# Autodesk Inventor assembly: Foot
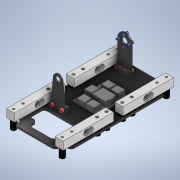
[picture p0: Inventor's stored thumbnail of the model, 180x180]
Saved by Autodesk Inventor 2022.3 (Build 263350000, 350)
## iProperties
Created: 2022-06-04
Part Number: Foot
Document SubType Name: Assembly
Designer: Masato Kubotera
Author: Masato Kubotera
## Documents named in this file (10)
- C:\Users\Masato\Documents\Inventor\CIT Brains\SUSTAINA-OP - mod\LowerBody\Foot\Foot.iam
- C:\Users\Masato\Documents\Inventor\CIT Brains\SUSTAINA-OP - mod\LowerBody\Foot\Foot_back_frame.ipt
- C:\Users\Masato\Documents\Inventor\CIT Brains\SUSTAINA-OP - mod\LowerBody\Foot\Foot_front_frame.ipt
- C:\Users\Masato\Documents\Inventor\CIT Brains\SUSTAINA-OP - mod\LowerBody\Foot\Foot_root_block.ipt
- C:\Users\Masato\Documents\Inventor\CIT Brains\SUSTAINA-OP - mod\LowerBody\Foot\Sole_frame.ipt
- C:\Users\Masato\Documents\Inventor\CIT Brains\SUSTAINA-OP - mod\ReadyMade\Screw\UC-0308.ipt
- C:\Users\Masato\Documents\Inventor\CIT Brains\SUSTAINA-OP - mod\ReadyMade\Screw\UC-2606.ipt
- C:\Users\Masato\Documents\Inventor\CIT Brains\SUSTAINA-OP - mod\LowerBody\Foot\LoadCell_unit.iam
- C:\Users\Masato\Documents\Inventor\CIT Brains\SUSTAINA-OP - mod\ReadyMade\Screw\FC-0515EB.ipt
- C:\Users\Masato\Documents\Inventor\CIT Brains\SUSTAINA-OP - mod\ReadyMade\ElectronicComponents\Quad-Load-Cell-Amplifier-to-RS-485-Conv-Module.ipt
## Components (30 placed, 9 different names)
1. Sole_frame:1 — 挿入:1, 挿入:2, 挿入:3, 挿入:4, 挿入:13, 挿入:14, 挿入:15, 挿入:16, 挿入:33, 挿入:34, 挿入:35, 挿入:36, 挿入:37, 挿入:38, 挿入:39, 挿入:40, 挿入:41, 挿入:42, 挿入:43, 挿入:44, 挿入:45, 挿入:46, 挿入:47, 挿入:48, 挿入:49, 挿入:50
2. Foot_front_frame:1 — 挿入:5, 挿入:6, メイト:1, メイト:2, 挿入:31, 挿入:32
3. Foot_back_frame:1 — 挿入:7, 挿入:8, 挿入:17, 挿入:18, 挿入:19, 挿入:20, 挿入:29, 挿入:30
4. Foot_root_block:1 — 挿入:1, 挿入:2, 挿入:5, 挿入:6
5. Foot_root_block:2 — 挿入:3, 挿入:4, 挿入:7, 挿入:8
6. UC-0308:5 — 挿入:32
7. UC-0308:6 — 挿入:31
8. UC-0308:7 — 挿入:29
9. UC-0308:8 — 挿入:30
10. UC-0308:1 — 挿入:13
11. UC-0308:2 — 挿入:14
12. UC-0308:3 — 挿入:15
13. UC-0308:4 — 挿入:16
14. UC-2606:1 — 挿入:17
15. UC-2606:2 — 挿入:18
16. UC-2606:3 — 挿入:19
17. UC-2606:4 — 挿入:20
18. LoadCell_unit:1 [sub-assembly] — 挿入:33, 挿入:34
19. LoadCell_unit:2 [sub-assembly] — 挿入:35, 挿入:36
20. LoadCell_unit:3 [sub-assembly] — 挿入:37, 挿入:38
21. LoadCell_unit:4 [sub-assembly] — 挿入:39, 挿入:40
22. FC-0515EB:1 — 挿入:41
23. FC-0515EB:2 — 挿入:42
24. FC-0515EB:3 — 挿入:43
25. FC-0515EB:4 — 挿入:44
26. FC-0515EB:5 — 挿入:45
27. FC-0515EB:6 — 挿入:46
28. FC-0515EB:7 — 挿入:47
29. FC-0515EB:8 — 挿入:48
30. Quad-Load-Cell-Amplifier-to-RS-485-Conv-Module:1 — 挿入:49, 挿入:50
## Relationships (40: Insert 38, Mate 2)
- メイト:1 [Mate]: Foot_front_frame:1
- メイト:2 [Mate]: Foot_front_frame:1
- 挿入:1 [Insert]: Sole_frame:1 ↔ Foot_root_block:1
- 挿入:2 [Insert]: Sole_frame:1 ↔ Foot_root_block:1
- 挿入:3 [Insert]: Sole_frame:1 ↔ Foot_root_block:2
- 挿入:4 [Insert]: Sole_frame:1 ↔ Foot_root_block:2
- 挿入:5 [Insert]: Foot_front_frame:1 ↔ Foot_root_block:1
- 挿入:6 [Insert]: Foot_front_frame:1 ↔ Foot_root_block:1
- 挿入:7 [Insert]: Foot_back_frame:1 ↔ Foot_root_block:2
- 挿入:8 [Insert]: Foot_back_frame:1 ↔ Foot_root_block:2
- 挿入:13 [Insert]: Sole_frame:1 ↔ UC-0308:1
- 挿入:14 [Insert]: Sole_frame:1 ↔ UC-0308:2
- 挿入:15 [Insert]: Sole_frame:1 ↔ UC-0308:3
- 挿入:16 [Insert]: Sole_frame:1 ↔ UC-0308:4
- 挿入:17 [Insert]: Foot_back_frame:1 ↔ UC-2606:1
- 挿入:18 [Insert]: Foot_back_frame:1 ↔ UC-2606:2
- 挿入:19 [Insert]: Foot_back_frame:1 ↔ UC-2606:3
- 挿入:20 [Insert]: Foot_back_frame:1 ↔ UC-2606:4
- 挿入:29 [Insert]: Foot_back_frame:1 ↔ UC-0308:7
- 挿入:30 [Insert]: Foot_back_frame:1 ↔ UC-0308:8
- 挿入:31 [Insert]: Foot_front_frame:1 ↔ UC-0308:6
- 挿入:32 [Insert]: Foot_front_frame:1 ↔ UC-0308:5
- 挿入:33 [Insert]: Sole_frame:1 ↔ LoadCell_unit:1
- 挿入:34 [Insert]: Sole_frame:1 ↔ LoadCell_unit:1
- 挿入:35 [Insert]: Sole_frame:1 ↔ LoadCell_unit:2
- 挿入:36 [Insert]: Sole_frame:1 ↔ LoadCell_unit:2
- 挿入:37 [Insert]: Sole_frame:1 ↔ LoadCell_unit:3
- 挿入:38 [Insert]: Sole_frame:1 ↔ LoadCell_unit:3
- 挿入:39 [Insert]: Sole_frame:1 ↔ LoadCell_unit:4
- 挿入:40 [Insert]: Sole_frame:1 ↔ LoadCell_unit:4
- 挿入:41 [Insert]: Sole_frame:1 ↔ FC-0515EB:1
- 挿入:42 [Insert]: Sole_frame:1 ↔ FC-0515EB:2
- 挿入:43 [Insert]: Sole_frame:1 ↔ FC-0515EB:3
- 挿入:44 [Insert]: Sole_frame:1 ↔ FC-0515EB:4
- 挿入:45 [Insert]: Sole_frame:1 ↔ FC-0515EB:5
- 挿入:46 [Insert]: Sole_frame:1 ↔ FC-0515EB:6
- 挿入:47 [Insert]: Sole_frame:1 ↔ FC-0515EB:7
- 挿入:48 [Insert]: Sole_frame:1 ↔ FC-0515EB:8
- 挿入:49 [Insert] (3 mm): Sole_frame:1 ↔ Quad-Load-Cell-Amplifier-to-RS-485-Conv-Module:1
- 挿入:50 [Insert] (3 mm): Sole_frame:1 ↔ Quad-Load-Cell-Amplifier-to-RS-485-Conv-Module:1
